# Autodesk Inventor assembly: Baugruppe_Montage_Ring_Hinten
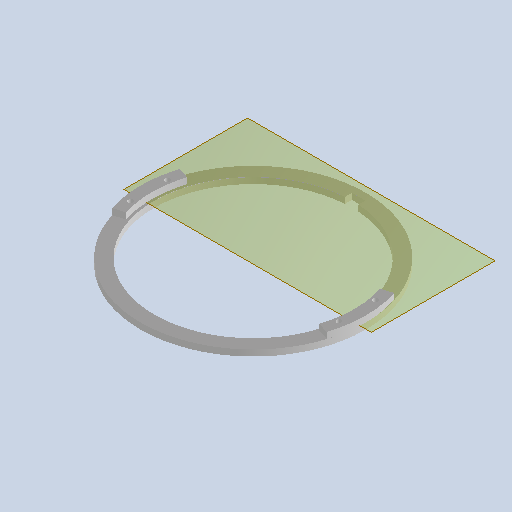
[picture p0: Inventor's stored thumbnail of the model, 512x512]
Saved by Autodesk Inventor 2022.2 (Build 262287010, 287A)
## iProperties
Created: 2024-01-10
Part Number: Baugruppe_Montage_Ring_Hinten
Document SubType Name: Assembly
Designer: ppovolni
Author: ppovolni
## Documents named in this file (5)
- D:\3_Local_Projekte\Weitere_Projekte\weitere_hw_projekte\Hallmesssonde - 8fach_Hallsensor\6_Entwurf Zylinderspule für Kalibrierung\Zylinderspule_Kalibrierung\CAD_Zylinderspule\Baugruppe_Montage_Ring_Hinten.iam
- D:\3_Local_Projekte\Weitere_Projekte\weitere_hw_projekte\Hallmesssonde - 8fach_Hallsensor\6_Entwurf Zylinderspule für Kalibrierung\Zylinderspule_Kalibrierung\CAD_Zylinderspule\Montage_Ring_Hinten_Teil1.ipt
- D:\3_Local_Projekte\Weitere_Projekte\weitere_hw_projekte\Hallmesssonde - 8fach_Hallsensor\6_Entwurf Zylinderspule für Kalibrierung\Zylinderspule_Kalibrierung\CAD_Zylinderspule\Montage_Ring_Hinten_Teil2.ipt
- D:\3_Local_Projekte\Weitere_Projekte\weitere_hw_projekte\Hallmesssonde - 8fach_Hallsensor\6_Entwurf Zylinderspule für Kalibrierung\Zylinderspule_Kalibrierung\CAD_Zylinderspule\Montage_Ring_Hinten_Aufdickung.ipt
- D:\3_Local_Projekte\Weitere_Projekte\weitere_hw_projekte\Hallmesssonde - 8fach_Hallsensor\6_Entwurf Zylinderspule für Kalibrierung\Zylinderspule_Kalibrierung\CAD_Zylinderspule\Montage_Ring_Hinten_Aufdickung_MIR.ipt
## Components (4 placed, 4 different names)
1. Montage_Ring_Hinten_Teil1:1 — Fluchtend:1, Passend:1, Passend:2, Fluchtend:2, Fluchtend:3
2. Montage_Ring_Hinten_Teil2:1 — Fluchtend:1, Passend:1, Passend:2
3. Montage_Ring_Hinten_Aufdickung:1 — Fluchtend:2, Fluchtend:3
4. Montage_Ring_Hinten_Aufdickung_MIR:1
## Relationships (5: Flush 3, Mate 2)
- Fluchtend:1 [Flush]: Montage_Ring_Hinten_Teil1:1 ↔ Montage_Ring_Hinten_Teil2:1
- Passend:1 [Mate]: Montage_Ring_Hinten_Teil1:1 ↔ Montage_Ring_Hinten_Teil2:1
- Passend:2 [Mate]: Montage_Ring_Hinten_Teil1:1 ↔ Montage_Ring_Hinten_Teil2:1
- Fluchtend:2 [Flush]: Montage_Ring_Hinten_Teil1:1 ↔ Montage_Ring_Hinten_Aufdickung:1
- Fluchtend:3 [Flush]: Montage_Ring_Hinten_Teil1:1 ↔ Montage_Ring_Hinten_Aufdickung:1
